# Autodesk Inventor assembly: 156
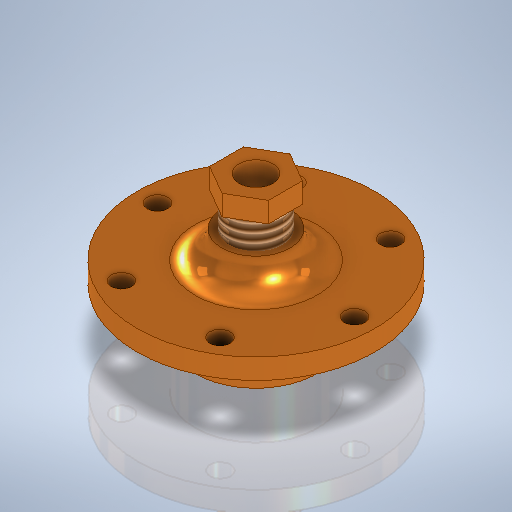
[picture p0: Inventor's stored thumbnail of the model, 512x512]
Saved by Autodesk Inventor 2025.1 (Build 291241000, 241)
## iProperties
Created: 2024-08-03
Part Number: 156
Document SubType Name: Assembly
Designer: ffogue
Author: ffogue
## Documents named in this file (3)
- C:\Projkete - Übungen\Freedom\156.iam
- C:\Projkete - Übungen\Freedom\156 part 2.ipt
- C:\Projkete - Übungen\Freedom\156.ipt
## Components (2 placed, 2 different names)
1. 156:1 — Mate:1, Insert:1
2. 156 part 2:1 — Mate:1, Insert:1
## Relationships (2: Mate 1, Insert 1)
- Mate:1: 156:1 ↔ 156 part 2:1
- Insert:1 (-3 mm): 156:1 ↔ 156 part 2:1
